# Autodesk Inventor assembly: MechanumChassis
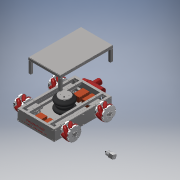
[picture p0: Inventor's stored thumbnail of the model, 180x180]
Saved by Autodesk Inventor 2018 (Build 220112000, 112)
## iProperties
Created: 2017-10-18
Part Number: MechanumChassis
Document SubType Name: Weldment
Designer: Bryce Richards
Mass: 42172.1 g
Surface Area: 44852.8 cm^2
Volume: 5448.29 cm^3
Density: 7.74044 g/cm^3
Weld Material: Steel, Mild, Welded
Author: Bryce Richards
## Documents named in this file (33)
- C:\Users\P136265\Documents\mecanum-cad\MechanumChassis.iam
- C:\Users\P136265\Documents\mecanum-cad\MecanumFrame2.iam
- C:\Users\P136265\Documents\mecanum-cad\PillowAssembly.iam
- C:\Users\P136265\Documents\Inventor\Content Center Files\R2018\en-US\AS 1110\AS 1110 - M8 x 60.ipt
- C:\Users\P136265\Documents\Inventor\Content Center Files\R2018\en-US\AS 1112 (2)\AS 1112 - M8  Type 5.ipt
- C:\Users\P136265\Documents\mecanum-cad\PillowPlate.ipt
- C:\Users\P136265\Documents\mecanum-cad\LiftPlate.iam
- C:\Users\P136265\Documents\mecanum-cad\AlignmentTube.ipt
- C:\Users\P136265\Documents\mecanum-cad\WheelShaft.ipt
- C:\Users\P136265\Documents\mecanum-cad\Mecanum_Assembly.iam
- C:\Users\P136265\Documents\Inventor\Content Center Files\R2018\en-US\ISO 4032(2)\ISO 4032 - M20 - ISO.ipt
- C:\Users\P136265\Documents\mecanum-cad\Cover_FrontRear.ipt
- C:\Users\P136265\Documents\mecanum-cad\Cover_LeftRight.ipt
- C:\Users\P136265\Documents\Inventor\Content Center Files\R2018\en-US\CNS 4373\CNS 4373 - M 4.ipt
- C:\Users\P136265\Documents\mecanum-cad\Cover_LiftSurface.ipt
- C:\Users\P136265\Documents\mecanum-cad\Compressor_PX06.ipt
- C:\Users\P136265\Documents\mecanum-cad\RestraintPlate.ipt
- C:\Users\P136265\Documents\Inventor\Content Center Files\R2018\en-US\AS 1420\AS 1420 - 1973 - M4 x 12.ipt
- C:\Users\P136265\Documents\mecanum-cad\Cover_Rear.ipt
- C:\Users\P136265\Documents\Inventor\Content Center Files\R2018\en-US\AS 1112 (2)\AS 1112 - M4  Type 5.ipt
- C:\Users\P136265\Documents\Inventor\Content Center Files\R2018\en-US\AS 1110\AS 1110 - M4 x 10.ipt
- C:\Users\P136265\Documents\mecanum-cad\LiftBase.ipt
- C:\Users\P136265\Documents\mecanum-cad\Firestone.ipt
- C:\Users\P136265\Documents\Inventor\Content Center Files\R2018\en-US\AS 1110\AS 1110 - M8 x 12.ipt
- C:\Users\P136265\Documents\mecanum-cad\Nema 23 Stepper Motor Bipolar L=56mm w Gear Ratio 41 Planetary Gearbox.ipt
- C:\Users\P136265\Documents\mecanum-cad\NP12-12FR Battery.ipt
- C:\Users\P136265\Documents\mecanum-cad\BatteryPlate.ipt
- C:\Users\P136265\Documents\mecanum-cad\MechanumChassis\AIP\FEA\cayefugld.fres
- C:\Users\P136265\Documents\mecanum-cad\MechanumChassis\AIP\FEA\cayefugao.fins
- C:\Users\P136265\Documents\mecanum-cad\MechanumChassis\AIP\FEA\cayefugao.fsat
- C:\Users\P136265\Documents\mecanum-cad\MechanumChassis\AIP\FEA\cayefugao.ftes
- C:\Users\P136265\Documents\mecanum-cad\MechanumChassis\AIP\FEA\cayefugao.fwiz
- C:\Users\P136265\Documents\mecanum-cad\MechanumChassis\AIP\FEA\cayefuglc.fmsh
## Components (135 placed, 26 different names)
1. MecanumFrame2:1 [sub-assembly] — Flush:2, Flush:6, Flush:7, Mate:56, Mate:69, Mate:70, Mate:71, Mate:90, Angle:5, Angle:6, Angle:7, Flush:10, Insert:17, Insert:18, Insert:19, Insert:20, Insert:21, Insert:22, Insert:23, Insert:24, Insert:25, Insert:26, Insert:27, Insert:28, Insert:29, Insert:30, Insert:31, Insert:32, Angle:8, Mate:209, Mate:210, Flush:11, Angle:9, Angle:10, Angle:11, Mate:211, Mate:212, Flush:12, Mate:213, Mate:214, Flush:13, Mate:215, Mate:216, Flush:14, Mate:234, Mate:235, Mate:236, Mate:237, Angle:29, Mate:263, Mate:265, Mate:266, Mate:267, Mate:268, Mate:269, Mate:270, Mate:271, Mate:273, Mate:275, Mate:277, Mate:279, Mate:281, Mate:283, Mate:285, Mate:287, Mate:289, Mate:291, Mate:293, Mate:295, Mate:297, Mate:299, Mate:301, Mate:303, Mate:305, Mate:307, Mate:309, Mate:353, Mate:354, Mate:355, Mate:386, Flush:32, Flush:33, Angle:34, Flush:34, Mate:395, Mate:396, Mate:397, Flush:35, Mate:398, Flush:36, Mate:399, Mate:400, Mate:402, Mate:403, Mate:405, Mate:406, Mate:408, Mate:409, Mate:410, Mate:411, Mate:412
2. PillowAssembly:1 [sub-assembly] — Mate:16, Mate:59, Mate:186, Mate:190, Mate:234
3. PillowAssembly:2 [sub-assembly] — Mate:13, Mate:62, Mate:178, Mate:180, Mate:235
4. PillowAssembly:3 [sub-assembly] — Mate:15, Mate:63, Mate:64, Mate:202, Mate:206, Mate:236
5. PillowAssembly:4 [sub-assembly] — Mate:51, Mate:52, Mate:53, Mate:194, Mate:196, Mate:237
6. PillowAssembly:5 [sub-assembly] — Mate:13, Flush:2, Mate:60, Mate:61, Mate:182, Mate:184, Mate:320, Flush:29, Mate:329
7. PillowAssembly:6 [sub-assembly] — Mate:15, Mate:65, Flush:10, Mate:204, Mate:208, Mate:317, Flush:27, Mate:327
8. PillowAssembly:7 [sub-assembly] — Flush:6, Mate:16, Mate:57, Mate:58, Mate:188, Mate:192, Mate:323, Flush:31, Mate:331
9. PillowAssembly:8 [sub-assembly] — Flush:7, Mate:51, Mate:54, Mate:198, Mate:200, Mate:313, Flush:25, Mate:325
10. PillowPlate:1 — Mate:52, Mate:53, Mate:54, Mate:56
11. PillowPlate:2 — Mate:57, Mate:58, Mate:59, Mate:71
12. PillowPlate:3 — Mate:60, Mate:61, Mate:62, Mate:70
13. PillowPlate:4 — Mate:63, Mate:64, Mate:65, Mate:69
14. LiftPlate:1 [sub-assembly] — Angle:29, Angle:30, Angle:31, Angle:32, Angle:33, Mate:263, Mate:311, Flush:22, Flush:23
15. AS 1110 - Metric M8 x 60:33 — Insert:17, Mate:179
16. AS 1110 - Metric M8 x 60:34 — Insert:18, Mate:177
17. AS 1110 - Metric M8 x 60:35 — Insert:19, Mate:183
18. AS 1110 - Metric M8 x 60:36 — Insert:20, Mate:181
19. AS 1110 - Metric M8 x 60:37 — Insert:21, Mate:187
20. AS 1110 - Metric M8 x 60:38 — Insert:22, Mate:191
21. AS 1110 - Metric M8 x 60:39 — Insert:23, Mate:189
22. AS 1110 - Metric M8 x 60:40 — Insert:24, Mate:185
23. AS 1110 - Metric M8 x 60:41 — Insert:25, Mate:199
24. AS 1110 - Metric M8 x 60:42 — Insert:26, Mate:197
25. AS 1110 - Metric M8 x 60:43 — Insert:27, Mate:195
26. AS 1110 - Metric M8 x 60:44 — Insert:28, Mate:193
27. AS 1110 - Metric M8 x 60:45 — Insert:29, Mate:201
28. AS 1110 - Metric M8 x 60:46 — Insert:30, Mate:203
29. AS 1110 - Metric M8 x 60:47 — Insert:31, Mate:207
30. AS 1110 - Metric M8 x 60:48 — Insert:32, Mate:205
31. AS 1112 (2) - Metric M8  Type 5:33 — Mate:177, Mate:178
32. AS 1112 (2) - Metric M8  Type 5:34 — Mate:179, Mate:180
33. AS 1112 (2) - Metric M8  Type 5:35 — Mate:181, Mate:182
34. AS 1112 (2) - Metric M8  Type 5:36 — Mate:183, Mate:184
35. AS 1112 (2) - Metric M8  Type 5:37 — Mate:185, Mate:186
36. AS 1112 (2) - Metric M8  Type 5:38 — Mate:187, Mate:188
37. AS 1112 (2) - Metric M8  Type 5:39 — Mate:189, Mate:190
38. AS 1112 (2) - Metric M8  Type 5:40 — Mate:191, Mate:192
39. AS 1112 (2) - Metric M8  Type 5:41 — Mate:193, Mate:194
40. AS 1112 (2) - Metric M8  Type 5:42 — Mate:195, Mate:196
41. AS 1112 (2) - Metric M8  Type 5:43 — Mate:197, Mate:198
42. AS 1112 (2) - Metric M8  Type 5:44 — Mate:199, Mate:200
43. AS 1112 (2) - Metric M8  Type 5:45 — Mate:201, Mate:202
44. AS 1112 (2) - Metric M8  Type 5:46 — Mate:203, Mate:204
45. AS 1112 (2) - Metric M8  Type 5:47 — Mate:205, Mate:206
46. AS 1112 (2) - Metric M8  Type 5:48 — Mate:207, Mate:208
47. AlignmentTube:1 — Angle:10, Mate:213, Mate:214, Flush:13, Angle:33
48. AlignmentTube:2 — Angle:8, Mate:209, Mate:210, Flush:11, Angle:31
49. AlignmentTube:3 — Angle:11, Mate:215, Mate:216, Flush:14, Angle:32
50. AlignmentTube:4 — Angle:9, Mate:211, Mate:212, Flush:12, Angle:30
51. Mecanum_Assembly:1 [sub-assembly] — Mate:318, Mate:319, Flush:28, Mate:344, Mate:345, Mate:346, Mate:351
52. Mecanum_Assembly:2 [sub-assembly] — Mate:321, Mate:322, Flush:30, Mate:341, Mate:342, Mate:343, Mate:349
53. Mecanum_Assembly:3 [sub-assembly] — Mate:315, Mate:316, Flush:26, Mate:338, Mate:339, Mate:340, Mate:347
54. Mecanum_Assembly:4 [sub-assembly] — Mate:312, Flush:24, Mate:314, Mate:333, Mate:334, Mate:335, Mate:336
55. Cover_FrontRear:1 — Mate:410, Mate:411, Mate:412
56. Cover_LeftRight:1 — Mate:265, Mate:266, Mate:267, Mate:272, Mate:274, Mate:276, Mate:278, Mate:280, Mate:282
57. Cover_LeftRight:2 — Mate:268, Mate:269, Mate:270, Mate:292, Mate:294, Mate:296, Mate:298, Mate:300, Mate:302
58. CNS 4373 M 4:1 — Mate:271, Mate:272
59. CNS 4373 M 4:2 — Mate:273, Mate:274
60. CNS 4373 M 4:3 — Mate:275, Mate:276
61. CNS 4373 M 4:4 — Mate:277, Mate:278
62. CNS 4373 M 4:5 — Mate:279, Mate:280
63. CNS 4373 M 4:6 — Mate:281, Mate:282
64. CNS 4373 M 4:7 — Mate:283
65. CNS 4373 M 4:8 — Mate:285
66. CNS 4373 M 4:9 — Mate:287
67. CNS 4373 M 4:10 — Mate:289
68. CNS 4373 M 4:11 — Mate:291, Mate:292
69. CNS 4373 M 4:12 — Mate:293, Mate:294
70. CNS 4373 M 4:13 — Mate:295, Mate:296
71. CNS 4373 M 4:14 — Mate:297, Mate:298
72. CNS 4373 M 4:15 — Mate:299, Mate:300
73. CNS 4373 M 4:16 — Mate:301, Mate:302
74. CNS 4373 M 4:17 — Mate:303
75. CNS 4373 M 4:18 — Mate:305
76. CNS 4373 M 4:19 — Mate:307
77. CNS 4373 M 4:20 — Mate:309
78. Cover_LiftSurface:1 — Mate:311, Flush:22, Flush:23
79. WheelShaft:1 — Mate:312, Flush:24, Mate:313, Flush:25, Mate:314, Mate:324
80. WheelShaft:2 — Mate:318, Mate:319, Flush:28, Mate:320, Flush:29, Mate:328
81. WheelShaft:3 — Mate:315, Mate:316, Flush:26, Mate:317, Flush:27, Mate:326
82. WheelShaft:4 — Mate:321, Mate:322, Flush:30, Mate:323, Flush:31, Mate:330, Mate:394
83. ISO 4032 M20:1 — Mate:324, Mate:325
84. ISO 4032 M20:2 — Mate:326, Mate:327
85. ISO 4032 M20:3 — Mate:328, Mate:329
86. ISO 4032 M20:4 — Mate:330, Mate:331
87. Compressor_PX06:1 — Mate:356, Mate:358, Mate:367, Mate:368, Mate:369, Mate:370, Mate:371, Mate:372, Mate:373, Mate:374, Mate:375, Mate:376, Mate:377
88. RestraintPlate:1 — Mate:333, Mate:334, Mate:335, Mate:337
89. RestraintPlate:2 — Mate:338, Mate:339, Mate:340, Mate:348
90. RestraintPlate:3 — Mate:341, Mate:342, Mate:343, Mate:350
91. RestraintPlate:4 — Mate:344, Mate:345, Mate:346, Mate:352
92. Cover_Rear:1 — Mate:353, Mate:354, Mate:355, Mate:356, Mate:358, Mate:367, Mate:368, Mate:369, Mate:379, Mate:381, Mate:383, Mate:385
93. AS 1110 - Metric M4 x 10:1 — Mate:370, Mate:371, Mate:378
94. AS 1110 - Metric M4 x 10:2 — Mate:372, Mate:373, Mate:384
95. AS 1110 - Metric M4 x 10:3 — Mate:374, Mate:375, Mate:380
96. AS 1110 - Metric M4 x 10:4 — Mate:376, Mate:377, Mate:382
97. AS 1112 (2) - Metric M4  Type 5:1 — Mate:378, Mate:379
98. AS 1112 (2) - Metric M4  Type 5:2 — Mate:380, Mate:381
99. AS 1112 (2) - Metric M4  Type 5:3 — Mate:382, Mate:383
100. AS 1112 (2) - Metric M4  Type 5:4 — Mate:384, Mate:385
101. LiftBase:1 — Mate:386, Flush:32, Flush:33, Mate:387, Mate:388, Mate:389, Mate:391, Mate:393
102. Firestone:1 — Mate:387, Mate:388, Mate:389, Mate:390, Mate:392
103. AS 1110 - Metric M8 x 12:1 — Mate:390, Mate:391
104. AS 1110 - Metric M8 x 12:2 — Mate:392, Mate:393
105. Nema 23 Stepper Motor Bipolar L=56mm w Gear Ratio 41 Planetary Gearbox:1 — Angle:34, Mate:394
106. NP12-12FR Battery:1 — Flush:34, Mate:395, Mate:396
107. BatteryPlate:1 — Mate:397, Flush:35, Mate:398, Mate:401
108. BatteryPlate:2 — Flush:36, Mate:399, Mate:400, Mate:404, Mate:407
109. NP12-12FR Battery:2 — Mate:401, Mate:402, Mate:403
110. NP12-12FR Battery:3 — Mate:404, Mate:405, Mate:406
111. NP12-12FR Battery:4 — Mate:407, Mate:408, Mate:409
112. AS 1420 - Metric M4 x 12:1 — Mate:336, Mate:337
113. AS 1420 - Metric M4 x 12:2
114. AS 1420 - Metric M4 x 12:3
115. AS 1420 - Metric M4 x 12:4
116. AS 1420 - Metric M4 x 12:5
117. AS 1420 - Metric M4 x 12:6
118. AS 1420 - Metric M4 x 12:7 — Mate:347, Mate:348
119. AS 1420 - Metric M4 x 12:8
120. AS 1420 - Metric M4 x 12:9
121. AS 1420 - Metric M4 x 12:10
122. AS 1420 - Metric M4 x 12:11
123. AS 1420 - Metric M4 x 12:12
124. AS 1420 - Metric M4 x 12:13 — Mate:349, Mate:350
125. AS 1420 - Metric M4 x 12:14
126. AS 1420 - Metric M4 x 12:15
127. AS 1420 - Metric M4 x 12:16
128. AS 1420 - Metric M4 x 12:17
129. AS 1420 - Metric M4 x 12:18
130. AS 1420 - Metric M4 x 12:19 — Mate:351, Mate:352
131. AS 1420 - Metric M4 x 12:20
132. AS 1420 - Metric M4 x 12:21
133. AS 1420 - Metric M4 x 12:22
134. AS 1420 - Metric M4 x 12:23
135. AS 1420 - Metric M4 x 12:24
## Component patterns: (6 elements, first: AS 1420 - Metric M4 x 12:1), (6 elements, first: AS 1420 - Metric M4 x 12:7), (6 elements, first: AS 1420 - Metric M4 x 12:13), (6 elements, first: AS 1420 - Metric M4 x 12:19)
## Relationships (248: Mate 196, Flush 23, Insert 16, Angle 13)
- Mate:13: PillowAssembly:2 ↔ PillowAssembly:5
- Flush:2: MecanumFrame2:1 ↔ PillowAssembly:5
- Mate:15: PillowAssembly:3 ↔ PillowAssembly:6
- Flush:6: MecanumFrame2:1 ↔ PillowAssembly:7
- Mate:16: PillowAssembly:1 ↔ PillowAssembly:7
- Flush:7: MecanumFrame2:1 ↔ PillowAssembly:8
- Mate:51: PillowAssembly:4 ↔ PillowAssembly:8
- Mate:52: PillowAssembly:4 ↔ PillowPlate:1
- Mate:53: PillowAssembly:4 ↔ PillowPlate:1
- Mate:54: PillowAssembly:8 ↔ PillowPlate:1
- Mate:56: MecanumFrame2:1 ↔ PillowPlate:1
- Mate:57: PillowAssembly:7 ↔ PillowPlate:2
- Mate:58: PillowAssembly:7 ↔ PillowPlate:2
- Mate:59: PillowAssembly:1 ↔ PillowPlate:2
- Mate:60: PillowAssembly:5 ↔ PillowPlate:3
- Mate:61: PillowAssembly:5 ↔ PillowPlate:3
- Mate:62: PillowAssembly:2 ↔ PillowPlate:3
- Mate:63: PillowAssembly:3 ↔ PillowPlate:4
- Mate:64: PillowAssembly:3 ↔ PillowPlate:4
- Mate:65: PillowAssembly:6 ↔ PillowPlate:4
- Mate:69: MecanumFrame2:1 ↔ PillowPlate:4
- Mate:70: MecanumFrame2:1 ↔ PillowPlate:3
- Mate:71: MecanumFrame2:1 ↔ PillowPlate:2
- Mate:90: MecanumFrame2:1
- Angle:5 (0 deg): MecanumFrame2:1
- Angle:6 (0 deg): MecanumFrame2:1
- Angle:7 (0 deg): MecanumFrame2:1
- Flush:10: MecanumFrame2:1 ↔ PillowAssembly:6
- Insert:17: MecanumFrame2:1 ↔ AS 1110 - Metric M8 x 60:33
- Insert:18: MecanumFrame2:1 ↔ AS 1110 - Metric M8 x 60:34
- Insert:19: MecanumFrame2:1 ↔ AS 1110 - Metric M8 x 60:35
- Insert:20: MecanumFrame2:1 ↔ AS 1110 - Metric M8 x 60:36
- Insert:21: MecanumFrame2:1 ↔ AS 1110 - Metric M8 x 60:37
- Insert:22: MecanumFrame2:1 ↔ AS 1110 - Metric M8 x 60:38
- Insert:23: MecanumFrame2:1 ↔ AS 1110 - Metric M8 x 60:39
- Insert:24: MecanumFrame2:1 ↔ AS 1110 - Metric M8 x 60:40
- Insert:25: MecanumFrame2:1 ↔ AS 1110 - Metric M8 x 60:41
- Insert:26: MecanumFrame2:1 ↔ AS 1110 - Metric M8 x 60:42
- Insert:27: MecanumFrame2:1 ↔ AS 1110 - Metric M8 x 60:43
- Insert:28: MecanumFrame2:1 ↔ AS 1110 - Metric M8 x 60:44
- Insert:29: MecanumFrame2:1 ↔ AS 1110 - Metric M8 x 60:45
- Insert:30: MecanumFrame2:1 ↔ AS 1110 - Metric M8 x 60:46
- Insert:31: MecanumFrame2:1 ↔ AS 1110 - Metric M8 x 60:47
- Insert:32: MecanumFrame2:1 ↔ AS 1110 - Metric M8 x 60:48
- Mate:177: AS 1110 - Metric M8 x 60:34 ↔ AS 1112 (2) - Metric M8  Type 5:33
- Mate:178: PillowAssembly:2 ↔ AS 1112 (2) - Metric M8  Type 5:33
- Mate:179: AS 1110 - Metric M8 x 60:33 ↔ AS 1112 (2) - Metric M8  Type 5:34
- Mate:180: PillowAssembly:2 ↔ AS 1112 (2) - Metric M8  Type 5:34
- Mate:181: AS 1110 - Metric M8 x 60:36 ↔ AS 1112 (2) - Metric M8  Type 5:35
- Mate:182: PillowAssembly:5 ↔ AS 1112 (2) - Metric M8  Type 5:35
- Mate:183: AS 1110 - Metric M8 x 60:35 ↔ AS 1112 (2) - Metric M8  Type 5:36
- Mate:184: PillowAssembly:5 ↔ AS 1112 (2) - Metric M8  Type 5:36
- Mate:185: AS 1110 - Metric M8 x 60:40 ↔ AS 1112 (2) - Metric M8  Type 5:37
- Mate:186: PillowAssembly:1 ↔ AS 1112 (2) - Metric M8  Type 5:37
- Mate:187: AS 1110 - Metric M8 x 60:37 ↔ AS 1112 (2) - Metric M8  Type 5:38
- Mate:188: PillowAssembly:7 ↔ AS 1112 (2) - Metric M8  Type 5:38
- Mate:189: AS 1110 - Metric M8 x 60:39 ↔ AS 1112 (2) - Metric M8  Type 5:39
- Mate:190: PillowAssembly:1 ↔ AS 1112 (2) - Metric M8  Type 5:39
- Mate:191: AS 1110 - Metric M8 x 60:38 ↔ AS 1112 (2) - Metric M8  Type 5:40
- Mate:192: PillowAssembly:7 ↔ AS 1112 (2) - Metric M8  Type 5:40
- Mate:193: AS 1110 - Metric M8 x 60:44 ↔ AS 1112 (2) - Metric M8  Type 5:41
- Mate:194: PillowAssembly:4 ↔ AS 1112 (2) - Metric M8  Type 5:41
- Mate:195: AS 1110 - Metric M8 x 60:43 ↔ AS 1112 (2) - Metric M8  Type 5:42
- Mate:196: PillowAssembly:4 ↔ AS 1112 (2) - Metric M8  Type 5:42
- Mate:197: AS 1110 - Metric M8 x 60:42 ↔ AS 1112 (2) - Metric M8  Type 5:43
- Mate:198: PillowAssembly:8 ↔ AS 1112 (2) - Metric M8  Type 5:43
- Mate:199: AS 1110 - Metric M8 x 60:41 ↔ AS 1112 (2) - Metric M8  Type 5:44
- Mate:200: PillowAssembly:8 ↔ AS 1112 (2) - Metric M8  Type 5:44
- Mate:201: AS 1110 - Metric M8 x 60:45 ↔ AS 1112 (2) - Metric M8  Type 5:45
- Mate:202: PillowAssembly:3 ↔ AS 1112 (2) - Metric M8  Type 5:45
- Mate:203: AS 1110 - Metric M8 x 60:46 ↔ AS 1112 (2) - Metric M8  Type 5:46
- Mate:204: PillowAssembly:6 ↔ AS 1112 (2) - Metric M8  Type 5:46
- Mate:205: AS 1110 - Metric M8 x 60:48 ↔ AS 1112 (2) - Metric M8  Type 5:47
- Mate:206: PillowAssembly:3 ↔ AS 1112 (2) - Metric M8  Type 5:47
- Mate:207: AS 1110 - Metric M8 x 60:47 ↔ AS 1112 (2) - Metric M8  Type 5:48
- Mate:208: PillowAssembly:6 ↔ AS 1112 (2) - Metric M8  Type 5:48
- Angle:8 (0 deg): MecanumFrame2:1 ↔ AlignmentTube:2
- Mate:209: MecanumFrame2:1 ↔ AlignmentTube:2
- Mate:210: MecanumFrame2:1 ↔ AlignmentTube:2
- Flush:11: MecanumFrame2:1 ↔ AlignmentTube:2
- Angle:9 (0 deg): MecanumFrame2:1 ↔ AlignmentTube:4
- Angle:10 (0 deg): MecanumFrame2:1 ↔ AlignmentTube:1
- Angle:11 (0 deg): MecanumFrame2:1 ↔ AlignmentTube:3
- Mate:211: MecanumFrame2:1 ↔ AlignmentTube:4
- Mate:212: MecanumFrame2:1 ↔ AlignmentTube:4
- Flush:12: MecanumFrame2:1 ↔ AlignmentTube:4
- Mate:213: MecanumFrame2:1 ↔ AlignmentTube:1
- Mate:214: MecanumFrame2:1 ↔ AlignmentTube:1
- Flush:13: MecanumFrame2:1 ↔ AlignmentTube:1
- Mate:215: MecanumFrame2:1 ↔ AlignmentTube:3
- Mate:216: MecanumFrame2:1 ↔ AlignmentTube:3
- Flush:14: MecanumFrame2:1 ↔ AlignmentTube:3
- Mate:234: MecanumFrame2:1 ↔ PillowAssembly:1
- Mate:235: MecanumFrame2:1 ↔ PillowAssembly:2
- Mate:236: MecanumFrame2:1 ↔ PillowAssembly:3
- Mate:237: MecanumFrame2:1 ↔ PillowAssembly:4
- Angle:29 (0 deg): MecanumFrame2:1 ↔ LiftPlate:1
- Angle:30 (0 deg): LiftPlate:1 ↔ AlignmentTube:4
- Angle:31 (0 deg): LiftPlate:1 ↔ AlignmentTube:2
- Angle:32 (0 deg): LiftPlate:1 ↔ AlignmentTube:3
- Angle:33 (0 deg): LiftPlate:1 ↔ AlignmentTube:1
- Mate:263: MecanumFrame2:1 ↔ LiftPlate:1
- Mate:265: MecanumFrame2:1 ↔ Cover_LeftRight:1
- Mate:266: MecanumFrame2:1 ↔ Cover_LeftRight:1
- Mate:267: MecanumFrame2:1 ↔ Cover_LeftRight:1
- Mate:268: MecanumFrame2:1 ↔ Cover_LeftRight:2
- Mate:269: MecanumFrame2:1 ↔ Cover_LeftRight:2
- Mate:270: MecanumFrame2:1 ↔ Cover_LeftRight:2
- Mate:271: MecanumFrame2:1 ↔ CNS 4373 M 4:1
- Mate:272: Cover_LeftRight:1 ↔ CNS 4373 M 4:1
- Mate:273: MecanumFrame2:1 ↔ CNS 4373 M 4:2
- Mate:274: Cover_LeftRight:1 ↔ CNS 4373 M 4:2
- Mate:275: MecanumFrame2:1 ↔ CNS 4373 M 4:3
- Mate:276: Cover_LeftRight:1 ↔ CNS 4373 M 4:3
- Mate:277: MecanumFrame2:1 ↔ CNS 4373 M 4:4
- Mate:278: Cover_LeftRight:1 ↔ CNS 4373 M 4:4
- Mate:279: MecanumFrame2:1 ↔ CNS 4373 M 4:5
- Mate:280: Cover_LeftRight:1 ↔ CNS 4373 M 4:5
- Mate:281: MecanumFrame2:1 ↔ CNS 4373 M 4:6
- Mate:282: Cover_LeftRight:1 ↔ CNS 4373 M 4:6
- Mate:283: MecanumFrame2:1 ↔ CNS 4373 M 4:7
- Mate:285: MecanumFrame2:1 ↔ CNS 4373 M 4:8
- Mate:287: MecanumFrame2:1 ↔ CNS 4373 M 4:9
- Mate:289: MecanumFrame2:1 ↔ CNS 4373 M 4:10
- Mate:291: MecanumFrame2:1 ↔ CNS 4373 M 4:11
- Mate:292: Cover_LeftRight:2 ↔ CNS 4373 M 4:11
- Mate:293: MecanumFrame2:1 ↔ CNS 4373 M 4:12
- Mate:294: Cover_LeftRight:2 ↔ CNS 4373 M 4:12
- Mate:295: MecanumFrame2:1 ↔ CNS 4373 M 4:13
- Mate:296: Cover_LeftRight:2 ↔ CNS 4373 M 4:13
- Mate:297: MecanumFrame2:1 ↔ CNS 4373 M 4:14
- Mate:298: Cover_LeftRight:2 ↔ CNS 4373 M 4:14
- Mate:299: MecanumFrame2:1 ↔ CNS 4373 M 4:15
- Mate:300: Cover_LeftRight:2 ↔ CNS 4373 M 4:15
- Mate:301: MecanumFrame2:1 ↔ CNS 4373 M 4:16
- Mate:302: Cover_LeftRight:2 ↔ CNS 4373 M 4:16
- Mate:303: MecanumFrame2:1 ↔ CNS 4373 M 4:17
- Mate:305: MecanumFrame2:1 ↔ CNS 4373 M 4:18
- Mate:307: MecanumFrame2:1 ↔ CNS 4373 M 4:19
- Mate:309: MecanumFrame2:1 ↔ CNS 4373 M 4:20
- Mate:311: LiftPlate:1 ↔ Cover_LiftSurface:1
- Flush:22 (3 mm): LiftPlate:1 ↔ Cover_LiftSurface:1
- Flush:23 (3 mm): LiftPlate:1 ↔ Cover_LiftSurface:1
- Mate:312: Mecanum_Assembly:4 ↔ WheelShaft:1
- Flush:24: Mecanum_Assembly:4 ↔ WheelShaft:1
- Mate:313: PillowAssembly:8 ↔ WheelShaft:1
- Flush:25 (-25 mm): PillowAssembly:8 ↔ WheelShaft:1
- Mate:314: Mecanum_Assembly:4 ↔ WheelShaft:1
- Mate:315: Mecanum_Assembly:3 ↔ WheelShaft:3
- Mate:316: Mecanum_Assembly:3 ↔ WheelShaft:3
- Flush:26: Mecanum_Assembly:3 ↔ WheelShaft:3
- Mate:317: PillowAssembly:6 ↔ WheelShaft:3
- Flush:27 (-25 mm): PillowAssembly:6 ↔ WheelShaft:3
- Mate:318: Mecanum_Assembly:1 ↔ WheelShaft:2
- Mate:319: Mecanum_Assembly:1 ↔ WheelShaft:2
- Flush:28: Mecanum_Assembly:1 ↔ WheelShaft:2
- Mate:320: PillowAssembly:5 ↔ WheelShaft:2
- Flush:29 (-25 mm): PillowAssembly:5 ↔ WheelShaft:2
- Mate:321: Mecanum_Assembly:2 ↔ WheelShaft:4
- Mate:322: Mecanum_Assembly:2 ↔ WheelShaft:4
- Flush:30: Mecanum_Assembly:2 ↔ WheelShaft:4
- Mate:323: PillowAssembly:7 ↔ WheelShaft:4
- Flush:31 (-25 mm): PillowAssembly:7 ↔ WheelShaft:4
- Mate:324: WheelShaft:1 ↔ ISO 4032 M20:1
- Mate:325: PillowAssembly:8 ↔ ISO 4032 M20:1
- Mate:326: WheelShaft:3 ↔ ISO 4032 M20:2
- Mate:327: PillowAssembly:6 ↔ ISO 4032 M20:2
- Mate:328: WheelShaft:2 ↔ ISO 4032 M20:3
- Mate:329: PillowAssembly:5 ↔ ISO 4032 M20:3
- Mate:330: WheelShaft:4 ↔ ISO 4032 M20:4
- Mate:331: PillowAssembly:7 ↔ ISO 4032 M20:4
- Mate:333: Mecanum_Assembly:4 ↔ RestraintPlate:1
- Mate:334: Mecanum_Assembly:4 ↔ RestraintPlate:1
- Mate:335: Mecanum_Assembly:4 ↔ RestraintPlate:1
- Mate:336: Mecanum_Assembly:4 ↔ AS 1420 - Metric M4 x 12:1
- Mate:337: RestraintPlate:1 ↔ AS 1420 - Metric M4 x 12:1
- Mate:338: Mecanum_Assembly:3 ↔ RestraintPlate:2
- Mate:339: Mecanum_Assembly:3 ↔ RestraintPlate:2
- Mate:340: Mecanum_Assembly:3 ↔ RestraintPlate:2
- Mate:341: Mecanum_Assembly:2 ↔ RestraintPlate:3
- Mate:342: Mecanum_Assembly:2 ↔ RestraintPlate:3
- Mate:343: Mecanum_Assembly:2 ↔ RestraintPlate:3
- Mate:344: Mecanum_Assembly:1 ↔ RestraintPlate:4
- Mate:345: Mecanum_Assembly:1 ↔ RestraintPlate:4
- Mate:346: Mecanum_Assembly:1 ↔ RestraintPlate:4
- Mate:347: Mecanum_Assembly:3 ↔ AS 1420 - Metric M4 x 12:7
- Mate:348: RestraintPlate:2 ↔ AS 1420 - Metric M4 x 12:7
- Mate:349: Mecanum_Assembly:2 ↔ AS 1420 - Metric M4 x 12:13
- Mate:350: RestraintPlate:3 ↔ AS 1420 - Metric M4 x 12:13
- Mate:351: Mecanum_Assembly:1 ↔ AS 1420 - Metric M4 x 12:19
- Mate:352: RestraintPlate:4 ↔ AS 1420 - Metric M4 x 12:19
- Mate:353: MecanumFrame2:1 ↔ Cover_Rear:1
- Mate:354: MecanumFrame2:1 ↔ Cover_Rear:1
- Mate:355: MecanumFrame2:1 ↔ Cover_Rear:1
- Mate:356: Compressor_PX06:1 ↔ Cover_Rear:1
- Mate:358: Compressor_PX06:1 ↔ Cover_Rear:1
- Mate:367: Compressor_PX06:1 ↔ Cover_Rear:1
- Mate:368: Compressor_PX06:1 ↔ Cover_Rear:1
- Mate:369: Compressor_PX06:1 ↔ Cover_Rear:1
- Mate:370: Compressor_PX06:1 ↔ AS 1110 - Metric M4 x 10:1
- Mate:371: Compressor_PX06:1 ↔ AS 1110 - Metric M4 x 10:1
- Mate:372: Compressor_PX06:1 ↔ AS 1110 - Metric M4 x 10:2
- Mate:373: Compressor_PX06:1 ↔ AS 1110 - Metric M4 x 10:2
- Mate:374: Compressor_PX06:1 ↔ AS 1110 - Metric M4 x 10:3
- Mate:375: Compressor_PX06:1 ↔ AS 1110 - Metric M4 x 10:3
- Mate:376: Compressor_PX06:1 ↔ AS 1110 - Metric M4 x 10:4
- Mate:377: Compressor_PX06:1 ↔ AS 1110 - Metric M4 x 10:4
- Mate:378: AS 1110 - Metric M4 x 10:1 ↔ AS 1112 (2) - Metric M4  Type 5:1
- Mate:379: Cover_Rear:1 ↔ AS 1112 (2) - Metric M4  Type 5:1
- Mate:380: AS 1110 - Metric M4 x 10:3 ↔ AS 1112 (2) - Metric M4  Type 5:2
- Mate:381: Cover_Rear:1 ↔ AS 1112 (2) - Metric M4  Type 5:2
- Mate:382: AS 1110 - Metric M4 x 10:4 ↔ AS 1112 (2) - Metric M4  Type 5:3
- Mate:383: Cover_Rear:1 ↔ AS 1112 (2) - Metric M4  Type 5:3
- Mate:384: AS 1110 - Metric M4 x 10:2 ↔ AS 1112 (2) - Metric M4  Type 5:4
- Mate:385: Cover_Rear:1 ↔ AS 1112 (2) - Metric M4  Type 5:4
- Mate:386: MecanumFrame2:1 ↔ LiftBase:1
- Flush:32 (2.5 mm): MecanumFrame2:1 ↔ LiftBase:1
- Flush:33 (2.5 mm): MecanumFrame2:1 ↔ LiftBase:1
- Mate:387: LiftBase:1 ↔ Firestone:1
- Mate:388: LiftBase:1 ↔ Firestone:1
- Mate:389: LiftBase:1 ↔ Firestone:1
- Mate:390: Firestone:1 ↔ AS 1110 - Metric M8 x 12:1
- Mate:391: LiftBase:1 ↔ AS 1110 - Metric M8 x 12:1
- Mate:392: Firestone:1 ↔ AS 1110 - Metric M8 x 12:2
- Mate:393: LiftBase:1 ↔ AS 1110 - Metric M8 x 12:2
- Angle:34 (0 deg): MecanumFrame2:1 ↔ Nema 23 Stepper Motor Bipolar L=56mm w Gear Ratio 41 Planetary Gearbox:1
- Mate:394: WheelShaft:4 ↔ Nema 23 Stepper Motor Bipolar L=56mm w Gear Ratio 41 Planetary Gearbox:1
- Flush:34: MecanumFrame2:1 ↔ NP12-12FR Battery:1
- Mate:395: MecanumFrame2:1 ↔ NP12-12FR Battery:1
- Mate:396: MecanumFrame2:1 ↔ NP12-12FR Battery:1
- Mate:397: MecanumFrame2:1 ↔ BatteryPlate:1
- Flush:35 (2.5 mm): MecanumFrame2:1 ↔ BatteryPlate:1
- Mate:398 (107.5 mm): MecanumFrame2:1 ↔ BatteryPlate:1
- Flush:36 (2.5 mm): MecanumFrame2:1 ↔ BatteryPlate:2
- Mate:399: MecanumFrame2:1 ↔ BatteryPlate:2
- Mate:400 (107.5 mm): MecanumFrame2:1 ↔ BatteryPlate:2
- Mate:401: BatteryPlate:1 ↔ NP12-12FR Battery:2
- Mate:402: MecanumFrame2:1 ↔ NP12-12FR Battery:2
- Mate:403: MecanumFrame2:1 ↔ NP12-12FR Battery:2
- Mate:404: BatteryPlate:2 ↔ NP12-12FR Battery:3
- Mate:405: MecanumFrame2:1 ↔ NP12-12FR Battery:3
- Mate:406: MecanumFrame2:1 ↔ NP12-12FR Battery:3
- Mate:407: BatteryPlate:2 ↔ NP12-12FR Battery:4
- Mate:408: MecanumFrame2:1 ↔ NP12-12FR Battery:4
- Mate:409: MecanumFrame2:1 ↔ NP12-12FR Battery:4
- Mate:410: MecanumFrame2:1 ↔ Cover_FrontRear:1
- Mate:411: MecanumFrame2:1 ↔ Cover_FrontRear:1
- Mate:412: MecanumFrame2:1 ↔ Cover_FrontRear:1
## Named parameters: sa_0 = 0, sa_1 = -3.88819e-08, sa_2 = 1e+06
note: some values were not read from the file. Shown as the stored number, unit unknown: "sa_0", "sa_1", "sa_2".
